# Autodesk Inventor assembly: AdaptadorBancoDePruebas
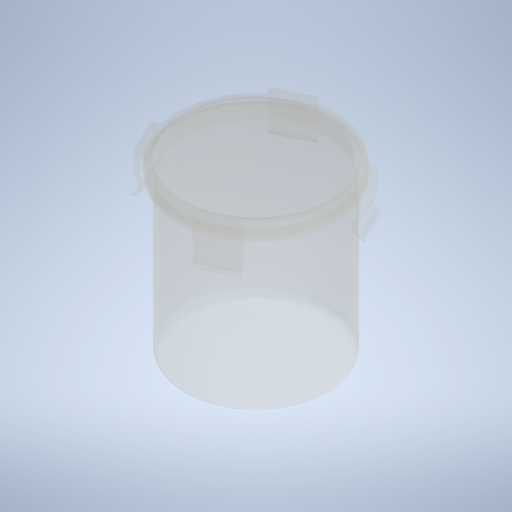
[picture p0: Inventor's stored thumbnail of the model, 512x512]
Saved by Autodesk Inventor 2024 (Build 280153000, 153)
## iProperties
Created: 2024-05-15
Part Number: AdaptadorBancoDePruebas
Document SubType Name: Assembly
Designer: alexa
Author: alexa
## Documents named in this file (3)
- C:\Users\alexa\OneDrive\Escritorio\Biogas\AdaptadorBancoDePruebas.iam
- C:\Users\alexa\OneDrive\Escritorio\Biogas\ContenedorTest.ipt
- C:\Users\alexa\OneDrive\Escritorio\Biogas\TapaContenedorTest.ipt
## Components (2 placed, 2 different names)
1. ContenedorTest:1 — Mate:1, Mate:2, Mate:3
2. TapaContenedorTest:1 — Mate:2, Mate:3
## Relationships (3: Mate 3)
- Mate:1: ContenedorTest:1
- Mate:2: ContenedorTest:1 ↔ TapaContenedorTest:1
- Mate:3: ContenedorTest:1 ↔ TapaContenedorTest:1
